# Autodesk Inventor assembly: Bev Chillah
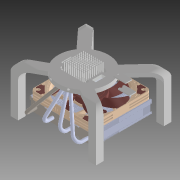
[picture p0: Inventor's stored thumbnail of the model, 180x180]
Saved by Autodesk Inventor 2020 (Build 240168000, 168)
## iProperties
Created: 2020-08-01
Part Number: Bev Chillah
Document SubType Name: Assembly
Designer: DDeGo
Author: DDeGo
## Documents named in this file (7)
- C:\Users\DDeGo\Documents\Drew\Projects\Bev Chillah\Bev Chillah.iam
- C:\Users\DDeGo\Documents\Drew\Projects\Bev Chillah\Noctua-NH-L12S.iam
- C:\Users\DDeGo\Documents\Drew\Projects\Bev Chillah\Bottom Bracket.ipt
- C:\Users\DDeGo\Documents\Drew\Projects\Bev Chillah\Peltier.ipt
- C:\Users\DDeGo\Documents\Drew\Projects\Bev Chillah\smol heatsink.ipt
- C:\Users\DDeGo\Documents\Drew\Projects\Bev Chillah\WindowInsert.ipt
- C:\Users\DDeGo\Documents\Drew\Projects\Bev Chillah\LED Backing.ipt
## Components (8 placed, 6 different names)
1. Noctua-NH-L12S:1 [sub-assembly] — Mate:1, Mate:5, Mate:6
2. Bottom Bracket:1 — Mate:3, Mate:4, Mate:5, Mate:6, Tangent:1, Mate:7, Mate:8, Mate:9, Mate:10, Mate:11, Mate:12
3. Peltier:1 — Mate:1, Flush:3, Flush:4, Mate:2
4. smol heatsink:1 — Flush:3, Flush:4, Mate:2, Mate:3, Mate:4, Tangent:1
5. WindowInsert:1 — Mate:7, Mate:11, Mate:12
6. WindowInsert:2 — Mate:8, Mate:9, Mate:10
7. LED Backing:1
8. LED Backing:2
## Relationships (15: Mate 12, Flush 2, Tangent 1)
- Mate:1: Noctua-NH-L12S:1 ↔ Peltier:1
- Flush:3: Peltier:1 ↔ smol heatsink:1
- Flush:4: Peltier:1 ↔ smol heatsink:1
- Mate:2: Peltier:1 ↔ smol heatsink:1
- Mate:3 (0.5 mm): Bottom Bracket:1 ↔ smol heatsink:1
- Mate:4 (0.5 mm): Bottom Bracket:1 ↔ smol heatsink:1
- Mate:5: Noctua-NH-L12S:1 ↔ Bottom Bracket:1
- Mate:6: Noctua-NH-L12S:1 ↔ Bottom Bracket:1
- Tangent:1: Bottom Bracket:1 ↔ smol heatsink:1
- Mate:7: Bottom Bracket:1 ↔ WindowInsert:1
- Mate:8: Bottom Bracket:1 ↔ WindowInsert:2
- Mate:9 (0.15 mm): Bottom Bracket:1 ↔ WindowInsert:2
- Mate:10 (0.15 mm): Bottom Bracket:1 ↔ WindowInsert:2
- Mate:11 (0.15 mm): Bottom Bracket:1 ↔ WindowInsert:1
- Mate:12 (0.15 mm): Bottom Bracket:1 ↔ WindowInsert:1
